# Autodesk Inventor assembly: ASY Beshkino_bio_tank
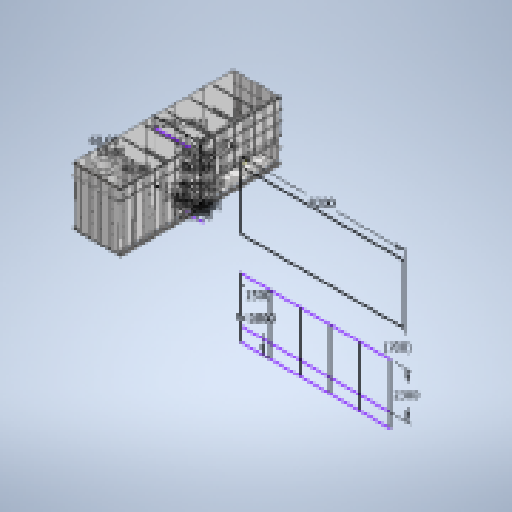
[picture p0: Inventor's stored thumbnail of the model, 512x512]
Saved by Autodesk Inventor 2025 (Build 290162010, 162A)
## iProperties
Created: 2024-07-21
Part Number: ASY Beshkino_bio_tank
Document SubType Name: Assembly
Designer: admin
Mass: 5.81287e+06 g
Surface Area: 2.77755e+06 cm^2
Volume: 3.12018e+06 cm^3
Density: 1.86299 g/cm^3
Author: admin
## Documents named in this file (46)
- C:\Users\DELL\YandexDisk-badmisterfox\домашниий пк\Inventor\BSH_Beshkino_bio_tank\ASY Beshkino_bio_tank.iam
- C:\Users\DELL\YandexDisk-badmisterfox\домашниий пк\Inventor\BSH_Beshkino_bio_tank\BSH 000 dim Beshkino_bio_tank.ipt
- C:\Users\DELL\YandexDisk-badmisterfox\домашниий пк\Inventor\BSH_Beshkino_bio_tank\BSH 011 floor.ipt
- C:\Users\DELL\YandexDisk-badmisterfox\домашниий пк\Inventor\BSH_Beshkino_bio_tank\BSH 021 rib floor.ipt
- C:\Users\DELL\YandexDisk-badmisterfox\домашниий пк\Inventor\BSH_Beshkino_bio_tank\BSH 022 rib board.ipt
- C:\Users\DELL\YandexDisk-badmisterfox\домашниий пк\Inventor\BSH_Beshkino_bio_tank\BSH 076 tube.ipt
- C:\Users\DELL\YandexDisk-badmisterfox\домашниий пк\Inventor\BSH_Beshkino_bio_tank\BSH 061 butt end.ipt
- C:\Users\DELL\YandexDisk-badmisterfox\домашниий пк\Inventor\BSH_Beshkino_bio_tank\BSH 041 board.ipt
- C:\Users\DELL\YandexDisk-badmisterfox\домашниий пк\Inventor\BSH_Beshkino_bio_tank\BSH 047 board.ipt
- C:\Users\DELL\YandexDisk-badmisterfox\домашниий пк\Inventor\BSH_Beshkino_bio_tank\BSH 045 back.ipt
- C:\Users\DELL\YandexDisk-badmisterfox\домашниий пк\Inventor\BSH_Beshkino_bio_tank\BSH 031 stringer floor.ipt
- C:\Users\DELL\YandexDisk-badmisterfox\домашниий пк\Inventor\BSH_Beshkino_bio_tank\BSH 036 stringer board 4.ipt
- C:\Users\DELL\YandexDisk-badmisterfox\домашниий пк\Inventor\BSH_Beshkino_bio_tank\BSH 032 stringer floor small.ipt
- C:\Users\DELL\YandexDisk-badmisterfox\домашниий пк\Inventor\BSH_Beshkino_bio_tank\BSH 039 stringer butt end in.ipt
- C:\Users\DELL\YandexDisk-badmisterfox\домашниий пк\Inventor\BSH_Beshkino_bio_tank\BSH 014 board cone.ipt
- C:\Users\DELL\YandexDisk-badmisterfox\домашниий пк\Inventor\BSH_Beshkino_bio_tank\BSH 051 sheet in.ipt
- C:\Users\DELL\YandexDisk-badmisterfox\домашниий пк\Inventor\BSH_Beshkino_bio_tank\BSH 071 amplifier in.ipt
- C:\Users\DELL\YandexDisk-badmisterfox\домашниий пк\Inventor\BSH_Beshkino_bio_tank\BSH 072 amplifier in.ipt
- C:\Users\DELL\YandexDisk-badmisterfox\домашниий пк\Inventor\BSH_Beshkino_bio_tank\BSH 012 floor.ipt
- C:\Users\DELL\YandexDisk-badmisterfox\домашниий пк\Inventor\BSH_Beshkino_bio_tank\BSH 016 cone.ipt
- C:\Users\DELL\YandexDisk-badmisterfox\домашниий пк\Inventor\BSH_Beshkino_bio_tank\BSH 013 floor.ipt
- C:\Users\DELL\YandexDisk-badmisterfox\домашниий пк\Inventor\BSH_Beshkino_bio_tank\BSH 015 board cone wall.ipt
- C:\Users\DELL\YandexDisk-badmisterfox\домашниий пк\Inventor\BSH_Beshkino_bio_tank\BSH 017 small detail floor.ipt
- C:\Users\DELL\YandexDisk-badmisterfox\домашниий пк\Inventor\BSH_Beshkino_bio_tank\BSH 038 stringer butt end.ipt
- C:\Users\DELL\YandexDisk-badmisterfox\домашниий пк\Inventor\BSH_Beshkino_bio_tank\BSH 053 sheet in.ipt
- C:\Users\DELL\YandexDisk-badmisterfox\домашниий пк\Inventor\BSH_Beshkino_bio_tank\BSH 044 board.ipt
- C:\Users\DELL\YandexDisk-badmisterfox\домашниий пк\Inventor\BSH_Beshkino_bio_tank\BSH 046 back.ipt
- C:\Users\DELL\YandexDisk-badmisterfox\домашниий пк\Inventor\BSH_Beshkino_bio_tank\BSH 042 board.ipt
- C:\Users\DELL\YandexDisk-badmisterfox\домашниий пк\Inventor\BSH_Beshkino_bio_tank\BSH 043 board.ipt
- C:\Users\DELL\YandexDisk-badmisterfox\домашниий пк\Inventor\BSH_Beshkino_bio_tank\BSH 052 sheet in.ipt
- C:\Users\DELL\YandexDisk-badmisterfox\домашниий пк\Inventor\BSH_Beshkino_bio_tank\BSH 023 rib butt end.ipt
- C:\Users\DELL\YandexDisk-badmisterfox\домашниий пк\Inventor\BSH_Beshkino_bio_tank\BSH 037 stringer board.ipt
- C:\Users\DELL\YandexDisk-badmisterfox\домашниий пк\Inventor\BSH_Beshkino_bio_tank\BSH 024 rib butt end in.ipt
- C:\Users\DELL\YandexDisk-badmisterfox\домашниий пк\Inventor\BSH_Beshkino_bio_tank\BSH 077 tube.ipt
- C:\Users\DELL\YandexDisk-badmisterfox\домашниий пк\Inventor\BSH_Beshkino_bio_tank\BSH 073 tube.ipt
- C:\Users\DELL\YandexDisk-badmisterfox\домашниий пк\Inventor\BSH_Beshkino_bio_tank\BSH 074 tube.ipt
- C:\Users\DELL\YandexDisk-badmisterfox\домашниий пк\Inventor\BSH_Beshkino_bio_tank\BSH 075 tube.ipt
- C:\Users\DELL\YandexDisk-badmisterfox\домашниий пк\Inventor\BSH_Beshkino_bio_tank\BSH 024 rib board short.ipt
- C:\Users\DELL\YandexDisk-badmisterfox\домашниий пк\Inventor\BSH_Beshkino_bio_tank\BSH 0363 stringer board 4.ipt
- C:\Users\DELL\YandexDisk-badmisterfox\домашниий пк\Inventor\BSH_Beshkino_bio_tank\BSH 022 rib floor 2.ipt
- C:\Users\DELL\YandexDisk-badmisterfox\домашниий пк\Inventor\BSH_Beshkino_bio_tank\BSH 033 stringer floor 3.ipt
- C:\Users\DELL\YandexDisk-badmisterfox\домашниий пк\Inventor\BSH_Beshkino_bio_tank\BSH 025 rib board cone.ipt
- C:\Users\DELL\YandexDisk-badmisterfox\домашниий пк\Inventor\BSH_Beshkino_bio_tank\ASY 080 barrel.iam
- C:\Users\DELL\YandexDisk-badmisterfox\домашниий пк\Inventor\BSH_Beshkino_bio_tank\BSH 0351 stringer board 3.ipt
- C:\Users\DELL\YandexDisk-badmisterfox\домашниий пк\Inventor\BSH_Beshkino_bio_tank\BSH 0341 stringer board 2.ipt
- C:\Users\DELL\YandexDisk-badmisterfox\домашниий пк\Inventor\BSH_Beshkino_bio_tank\BSH 014 board cone_CPY.ipt
## Components (129 placed, 48 different names)
1. BSH 000 dim Beshkino_bio_tank:1
2. BSH 076 tube:1 — Mate:1, Rigid:1, Mate:3, Mate:119, Flush:121, Flush:122, Mate:121, Flush:123
3. BSH 076 tube:2 — Mate:2, Rigid:1, Mate:4, Flush:3, Flush:4, Flush:124, Mate:132, Flush:128
4. BSH 011 floor:1 — Rigid:5, Rigid:83, Mate:77, Flush:18, Flush:19
5. BSH 011 floor:2 — Rigid:5, Rigid:82
6. BSH 011 floor:3 — Mate:5, Mate:6, Mate:7, Flush:4, Mate:10, Flush:5, Flush:11, Rigid:82, Mate:74, Mate:133
7. BSH 061 butt end:1 — Mate:10, Flush:5, Mate:11, Rigid:11, Mate:73, Mate:108, Mate:135, Flush:131, Mate:136
8. BSH 047 board:1 — Flush:11, Mate:73, Mate:74, Rigid:104, Mate:127, Flush:125, Flush:126, Mate:128, Flush:127
9. BSH 061 butt end:2 — Rigid:11, Rigid:53
10. BSH 021 rib floor:1 — Mate:4, Flush:3, Mate:5, Mate:6, Rigid:9, Rigid:109, Rigid:118, Rigid:122, Mate:120, Rigid:156
11. BSH 061 butt end:3 — Mate:113
12. BSH 061 butt end:4 — Rigid:53, Flush:112
13. BSH 014 board cone:1 — Mate:26, Rigid:57, Mate:30, Mate:80, Mate:83
14. BSH 061 butt end:5 — Mate:26, Mate:30, Mate:84, Flush:21, Mate:94, Mate:141
15. BSH 061 butt end:6 — Flush:8, Mate:40, Mate:111, Mate:137, Mate:138
16. BSH 014 board cone:2 — Rigid:57, Angle:1, Mate:49, Mate:50, Mate:64, Mate:71
17. BSH 036 stringer board 4:4 — Rigid:141
18. BSH 037 stringer board:1 — Rigid:141, Rigid:142
19. BSH 0363 stringer board 4:1 — Rigid:142, Rigid:143
20. BSH 051 sheet in:1 — Mate:84, Rigid:108, Mate:88, Mate:89, Mate:90, Mate:91, Mate:123
21. BSH 012 floor:1 — Rigid:66, Mate:42, Angle:1, Mate:49, Rigid:83, Mate:72, Mate:87
22. BSH 016 cone:1 — Mate:42, Mate:50, Mate:90
23. BSH 047 board:2 — Rigid:139
24. BSH 012 floor:2 — Rigid:66, Rigid:67, Mate:63, Mate:78, Mate:122
25. BSH 013 floor:1 — Rigid:67, Mate:40, Mate:81
26. BSH 045 back:1 — Rigid:90, Rigid:103
27. BSH 015 board cone wall:1 — Mate:71, Mate:72, Mate:85, Mate:86
28. BSH 017 small detail floor:1 — Mate:77, Flush:18, Flush:19
29. BSH 038 stringer butt end:1 — Mate:107, Mate:108, Rigid:128, Rigid:129, Rigid:130, Rigid:131
30. BSH 016 cone:2 — Mate:63, Mate:64, Mate:91
31. BSH 022 rib board:2 — Rigid:137, Mate:117, Flush:117
32. BSH 016 cone:3 — Mate:78, Mate:80, Mate:88
33. BSH 016 cone:4 — Mate:81, Mate:83, Mate:89
34. BSH 053 sheet in:1 — Rigid:107
35. BSH 044 board:1 — Rigid:90, Mate:85, Rigid:106
36. BSH 046 back:1 — Rigid:103, Flush:21, Mate:96, Flush:132, Mate:139
37. BSH 042 board:1 — Rigid:104, Rigid:105
38. BSH 043 board:1 — Rigid:105, Rigid:106
39. BSH 052 sheet in:1 — Rigid:107, Rigid:108, Mate:86, Mate:87
40. BSH 031 stringer floor:1 — Rigid:109, Rigid:147
41. BSH 032 stringer floor small:1 — Mate:131, Rigid:146
42. BSH 031 stringer floor:4 — Rigid:118
43. BSH 031 stringer floor:7 — Rigid:122
44. BSH 031 stringer floor:12 — Rigid:156
45. BSH 023 rib butt end:1 — Rigid:128, Mate:130
46. BSH 023 rib butt end:2 — Rigid:129
47. BSH 023 rib butt end:3 — Rigid:130
48. BSH 023 rib butt end:4 — Rigid:131
49. BSH 023 rib butt end:5
50. BSH 023 rib butt end:6
51. BSH 023 rib butt end:7
52. BSH 023 rib butt end:8 — Flush:129
53. BSH 022 rib board:3 — Rigid:138, Mate:128, Mate:129, Flush:127, Rigid:143
54. BSH 022 rib board:4 — Rigid:137
55. BSH 077 tube:1 — Mate:119, Flush:121, Flush:122, Mate:120, Mate:130
56. BSH 077 tube:2 — Mate:121, Flush:123, Flush:124, Mate:131, Flush:129
57. BSH 073 tube:1 — Mate:122, Mate:123, Mate:124
58. BSH 074 tube:1 — Mate:135, Flush:131, Mate:136
59. BSH 075 tube:2 — Mate:127, Flush:125, Flush:126, Mate:129, Mate:140
60. BSH 033 stringer floor 3:1 — Rigid:147
61. BSH 025 rib board cone:1 — Flush:130, Mate:134
62. ASY 080 barrel:1 [sub-assembly] — Mate:133
63. BSH 0351 stringer board 3:1 — Rigid:148
64. BSH 0341 stringer board 2:1 — Rigid:149
65. BSH 042 stringer floor:2 — Rigid:150
66. BSH 042 stringer floor:3 — Rigid:151
67. BSH 042 stringer floor:4 — Rigid:152
68. BSH 033 stringer floor 3:2 — Rigid:154
69. BSH 033 stringer floor 3:3 — Rigid:153
70. BSH 033 stringer floor 3:4 — Rigid:155
71. BSH 051 water tray:1 — Mate:139, Mate:140, Mate:141
72. BSH 041 board:1 — Mate:117, Flush:117, Rigid:139
73. BSH 041 board:2
74. BSH 041 board:3
75. BSH 041 board:4
76. BSH 041 board:5 — Mate:137, Flush:132, Mate:138
77. BSH 071 amplifier in:1 — Flush:22, Mate:94, Mate:96, Flush:24, Mate:97, Mate:124
78. BSH 072 amplifier in:1 — Flush:22, Mate:93, Flush:24
79. BSH 071 amplifier in:2
80. BSH 072 amplifier in:2
81. BSH 071 amplifier in:3
82. BSH 072 amplifier in:3
83. BSH 071 amplifier in:4
84. BSH 072 amplifier in:4
85. BSH 071 amplifier in:5
86. BSH 072 amplifier in:5
87. BSH 039 stringer butt end in:1 — Mate:23, Flush:112, Mate:113, Rigid:140
88. BSH 039 stringer butt end in:2
89. BSH 039 stringer butt end in:3
90. BSH 039 stringer butt end in:4
91. BSH 039 stringer butt end in:5
92. BSH 024 rib butt end in:1 — Rigid:140
93. BSH 024 rib butt end in:2
94. BSH 024 rib butt end in:3
95. BSH 024 rib butt end in:4
96. BSH 022 rib board:1 — Rigid:138
97. BSH 022 rib 2:36
98. BSH 022 rib 2:37
99. BSH 022 rib 2:38
100. BSH 022 rib 2:39
101. BSH 022 rib 2:40
102. BSH 022 rib 2:41
103. BSH 022 rib 2:42
104. BSH 022 rib 2:43 — Rigid:144
105. BSH 024 rib board short:1 — Rigid:144, Flush:130, Mate:134
106. BSH 024 rib board short:2
107. BSH 024 rib board short:3
108. BSH 024 rib board short:4
109. BSH 024 rib board short:5
110. BSH 024 rib board short:6 — Rigid:148, Rigid:149
111. BSH 021 rib floor:2 — Rigid:9
112. BSH 020 rib 1:4
113. BSH 020 rib 1:5
114. BSH 020 rib 1:6
115. BSH 020 rib 1:7 — Rigid:145
116. BSH 022 rib floor 2:1 — Rigid:146, Mate:132, Flush:128, Rigid:150, Rigid:151, Rigid:152
117. BSH 022 rib floor 2:2
118. BSH 022 rib floor 2:3
119. BSH 022 rib floor 2:4
120. BSH 022 rib floor 2:5
121. BSH 022 rib floor 2:6
122. BSH 020 rib 1:8 — Rigid:145
123. BSH 020 rib 1:9
124. BSH 020 rib 1:10
125. BSH 020 rib 1:11 — Rigid:153, Rigid:154, Rigid:155
126. BSH 038 stringer butt end:2 — Flush:111, Mate:111
127. BSH 038 stringer butt end:3
128. BSH 038 stringer butt end:4
129. BSH 038 stringer butt end:5
## Component patterns: (5 elements, first: BSH 041 board:1), (5 elements, first: BSH 071 amplifier in:1 + BSH 072 amplifier in:1), (5 elements, first: BSH 039 stringer butt end in:1), (4 elements, first: BSH 024 rib butt end in:1), (9 elements, first: BSH 022 rib board:1), (6 elements, first: BSH 024 rib board short:1), (5 elements, first: BSH 021 rib floor:2), (6 elements, first: BSH 022 rib floor 2:1), (4 elements, first: BSH 020 rib 1:8), (4 elements, first: BSH 038 stringer butt end:2)
## Relationships (141: Mate 65, WeldJoint 50, Flush 25, Angle 1)
- Mate:1: BSH 076 tube:1
- Mate:2: BSH 076 tube:2
- Rigid:1 [WeldJoint] (-2400 mm): BSH 076 tube:1 ↔ BSH 076 tube:2
- Mate:3: BSH 076 tube:1
- Mate:4: BSH 076 tube:2 ↔ BSH 021 rib floor:1
- Flush:3: BSH 076 tube:2 ↔ BSH 021 rib floor:1
- Mate:5: BSH 011 floor:3 ↔ BSH 021 rib floor:1
- Mate:6: BSH 011 floor:3 ↔ BSH 021 rib floor:1
- Rigid:5 [WeldJoint]: BSH 011 floor:1 ↔ BSH 011 floor:2
- Mate:7: BSH 011 floor:3
- Flush:4: BSH 076 tube:2 ↔ BSH 011 floor:3
- Rigid:9 [WeldJoint] (-500 mm): BSH 021 rib floor:1 ↔ BSH 021 rib floor:2
- Mate:10: BSH 011 floor:3 ↔ BSH 061 butt end:1
- Flush:5 (10 mm): BSH 011 floor:3 ↔ BSH 061 butt end:1
- Mate:11: BSH 061 butt end:1
- Rigid:11 [WeldJoint]: BSH 061 butt end:1 ↔ BSH 061 butt end:2
- Mate:23: BSH 039 stringer butt end in:1
- [WeldJoint]: BSH 061 butt end:3 ↔ BSH 061 butt end:4
- Rigid:53 [WeldJoint] (1500 mm): BSH 061 butt end:2 ↔ BSH 061 butt end:4
- [WeldJoint]: BSH 061 butt end:5 ↔ BSH 061 butt end:6
- Flush:8: BSH 061 butt end:6
- Mate:26: BSH 014 board cone:1 ↔ BSH 061 butt end:5
- Rigid:57 [WeldJoint]: BSH 014 board cone:1 ↔ BSH 014 board cone:2
- Mate:30: BSH 014 board cone:1 ↔ BSH 061 butt end:5
- Flush:11: BSH 011 floor:3 ↔ BSH 047 board:1
- Rigid:66 [WeldJoint]: BSH 012 floor:1 ↔ BSH 012 floor:2
- Rigid:67 [WeldJoint]: BSH 012 floor:2 ↔ BSH 013 floor:1
- Mate:40: BSH 061 butt end:6 ↔ BSH 013 floor:1
- Mate:42: BSH 012 floor:1 ↔ BSH 016 cone:1
- Angle:1 (132 deg): BSH 014 board cone:2 ↔ BSH 012 floor:1
- Mate:49: BSH 014 board cone:2 ↔ BSH 012 floor:1
- Mate:50: BSH 014 board cone:2 ↔ BSH 016 cone:1
- Mate:63: BSH 012 floor:2 ↔ BSH 016 cone:2
- Mate:64: BSH 014 board cone:2 ↔ BSH 016 cone:2
- Rigid:82 [WeldJoint]: BSH 011 floor:2 ↔ BSH 011 floor:3
- Rigid:83 [WeldJoint]: BSH 011 floor:1 ↔ BSH 012 floor:1
- Mate:71: BSH 014 board cone:2 ↔ BSH 015 board cone wall:1
- Mate:72: BSH 012 floor:1 ↔ BSH 015 board cone wall:1
- Mate:73: BSH 061 butt end:1 ↔ BSH 047 board:1
- Mate:74: BSH 011 floor:3 ↔ BSH 047 board:1
- Mate:77: BSH 011 floor:1 ↔ BSH 017 small detail floor:1
- Flush:18: BSH 011 floor:1 ↔ BSH 017 small detail floor:1
- Flush:19: BSH 011 floor:1 ↔ BSH 017 small detail floor:1
- Mate:78: BSH 012 floor:2 ↔ BSH 016 cone:3
- Mate:80: BSH 014 board cone:1 ↔ BSH 016 cone:3
- Mate:81: BSH 013 floor:1 ↔ BSH 016 cone:4
- Mate:83: BSH 014 board cone:1 ↔ BSH 016 cone:4
- Mate:84: BSH 061 butt end:5 ↔ BSH 051 sheet in:1
- Rigid:90 [WeldJoint]: BSH 045 back:1 ↔ BSH 044 board:1
- Mate:85: BSH 015 board cone wall:1 ↔ BSH 044 board:1
- Rigid:103 [WeldJoint]: BSH 045 back:1 ↔ BSH 046 back:1
- Rigid:104 [WeldJoint]: BSH 047 board:1 ↔ BSH 042 board:1
- Rigid:105 [WeldJoint]: BSH 042 board:1 ↔ BSH 043 board:1
- Rigid:106 [WeldJoint]: BSH 044 board:1 ↔ BSH 043 board:1
- Flush:21 (10 mm): BSH 061 butt end:5 ↔ BSH 046 back:1
- Rigid:107 [WeldJoint]: BSH 053 sheet in:1 ↔ BSH 052 sheet in:1
- Rigid:108 [WeldJoint]: BSH 051 sheet in:1 ↔ BSH 052 sheet in:1
- Mate:86: BSH 015 board cone wall:1 ↔ BSH 052 sheet in:1
- Mate:87: BSH 012 floor:1 ↔ BSH 052 sheet in:1
- Mate:88: BSH 051 sheet in:1 ↔ BSH 016 cone:3
- Mate:89: BSH 051 sheet in:1 ↔ BSH 016 cone:4
- Mate:90: BSH 051 sheet in:1 ↔ BSH 016 cone:1
- Mate:91: BSH 051 sheet in:1 ↔ BSH 016 cone:2
- Flush:22: BSH 071 amplifier in:1 ↔ BSH 072 amplifier in:1
- Mate:93: BSH 072 amplifier in:1
- Mate:94 (1000 mm): BSH 061 butt end:5 ↔ BSH 071 amplifier in:1
- Rigid:109 [WeldJoint] (2 mm): BSH 021 rib floor:1 ↔ BSH 031 stringer floor:1
- Rigid:118 [WeldJoint] (2 mm): BSH 021 rib floor:1 ↔ BSH 031 stringer floor:4
- Rigid:122 [WeldJoint] (2 mm): BSH 021 rib floor:1 ↔ BSH 031 stringer floor:7
- Mate:96 (100 mm): BSH 046 back:1 ↔ BSH 071 amplifier in:1
- Flush:24 (1000 mm): BSH 071 amplifier in:1 ↔ BSH 072 amplifier in:1
- Mate:97: BSH 071 amplifier in:1
- Mate:107: BSH 038 stringer butt end:1
- Mate:108: BSH 061 butt end:1 ↔ BSH 038 stringer butt end:1
- Rigid:128 [WeldJoint] (2 mm): BSH 038 stringer butt end:1 ↔ BSH 023 rib butt end:1
- Rigid:129 [WeldJoint] (2 mm): BSH 038 stringer butt end:1 ↔ BSH 023 rib butt end:2
- Rigid:130 [WeldJoint] (2 mm): BSH 038 stringer butt end:1 ↔ BSH 023 rib butt end:3
- Rigid:131 [WeldJoint] (2 mm): BSH 038 stringer butt end:1 ↔ BSH 023 rib butt end:4
- [WeldJoint] (2 mm): BSH 023 rib butt end:5 ↔ BSH 038 stringer butt end:2
- [WeldJoint] (2 mm): BSH 023 rib butt end:6 ↔ BSH 038 stringer butt end:2
- [WeldJoint] (2 mm): BSH 023 rib butt end:7 ↔ BSH 038 stringer butt end:2
- [WeldJoint] (2 mm): BSH 023 rib butt end:8 ↔ BSH 038 stringer butt end:2
- Flush:111: BSH 038 stringer butt end:2
- Mate:111: BSH 061 butt end:6 ↔ BSH 038 stringer butt end:2
- Flush:112 (171.5 mm): BSH 061 butt end:4 ↔ BSH 039 stringer butt end in:1
- Mate:113: BSH 061 butt end:3 ↔ BSH 039 stringer butt end in:1
- Rigid:137 [WeldJoint] (-436 mm): BSH 022 rib board:2 ↔ BSH 022 rib board:4
- Mate:117: BSH 022 rib board:2 ↔ BSH 041 board:1
- Flush:117 (-218 mm): BSH 022 rib board:2 ↔ BSH 041 board:1
- Rigid:138 [WeldJoint] (-500 mm): BSH 022 rib board:3 ↔ BSH 022 rib board:1
- Rigid:139 [WeldJoint]: BSH 047 board:2 ↔ BSH 041 board:1
- Rigid:140 [WeldJoint] (2 mm): BSH 039 stringer butt end in:1 ↔ BSH 024 rib butt end in:1
- Mate:119: BSH 076 tube:1 ↔ BSH 077 tube:1
- Flush:121: BSH 076 tube:1 ↔ BSH 077 tube:1
- Flush:122: BSH 076 tube:1 ↔ BSH 077 tube:1
- Mate:120 (117 mm): BSH 021 rib floor:1 ↔ BSH 077 tube:1
- Mate:121: BSH 076 tube:1 ↔ BSH 077 tube:2
- Flush:123: BSH 076 tube:1 ↔ BSH 077 tube:2
- Flush:124: BSH 076 tube:2 ↔ BSH 077 tube:2
- Mate:122: BSH 012 floor:2 ↔ BSH 073 tube:1
- Mate:123: BSH 051 sheet in:1 ↔ BSH 073 tube:1
- Mate:124: BSH 073 tube:1 ↔ BSH 071 amplifier in:1
- Rigid:141 [WeldJoint]: BSH 036 stringer board 4:4 ↔ BSH 037 stringer board:1
- Mate:127: BSH 047 board:1 ↔ BSH 075 tube:2
- Flush:125: BSH 047 board:1 ↔ BSH 075 tube:2
- Flush:126 (-40 mm): BSH 047 board:1 ↔ BSH 075 tube:2
- Mate:128: BSH 047 board:1 ↔ BSH 022 rib board:3
- Mate:129: BSH 022 rib board:3 ↔ BSH 075 tube:2
- Flush:127 (213.5 mm): BSH 047 board:1 ↔ BSH 022 rib board:3
- Rigid:142 [WeldJoint]: BSH 037 stringer board:1 ↔ BSH 0363 stringer board 4:1
- Rigid:143 [WeldJoint] (2 mm): BSH 0363 stringer board 4:1 ↔ BSH 022 rib board:3
- Rigid:144 [WeldJoint] (500 mm): BSH 022 rib 2:43 ↔ BSH 024 rib board short:1
- Mate:130: BSH 023 rib butt end:1 ↔ BSH 077 tube:1
- Mate:131: BSH 032 stringer floor small:1 ↔ BSH 077 tube:2
- Rigid:145 [WeldJoint] (500 mm): BSH 020 rib 1:7 ↔ BSH 020 rib 1:8
- Rigid:146 [WeldJoint] (2 mm): BSH 032 stringer floor small:1 ↔ BSH 022 rib floor 2:1
- Mate:132: BSH 076 tube:2 ↔ BSH 022 rib floor 2:1
- Flush:128: BSH 076 tube:2 ↔ BSH 022 rib floor 2:1
- Rigid:147 [WeldJoint] (-10 mm): BSH 031 stringer floor:1 ↔ BSH 033 stringer floor 3:1
- Flush:129: BSH 023 rib butt end:8 ↔ BSH 077 tube:2
- Mate:133: BSH 011 floor:3 ↔ ASY 080 barrel:1
- Flush:130: BSH 025 rib board cone:1 ↔ BSH 024 rib board short:1
- Mate:134: BSH 025 rib board cone:1 ↔ BSH 024 rib board short:1
- Rigid:148 [WeldJoint] (2 mm): BSH 0351 stringer board 3:1 ↔ BSH 024 rib board short:6
- Rigid:149 [WeldJoint] (2 mm): BSH 0341 stringer board 2:1 ↔ BSH 024 rib board short:6
- Mate:135: BSH 061 butt end:1 ↔ BSH 074 tube:1
- Flush:131: BSH 061 butt end:1 ↔ BSH 074 tube:1
- Mate:136: BSH 061 butt end:1 ↔ BSH 074 tube:1
- Rigid:150 [WeldJoint] (2 mm): BSH 042 stringer floor:2 ↔ BSH 022 rib floor 2:1
- Rigid:151 [WeldJoint] (2 mm): BSH 042 stringer floor:3 ↔ BSH 022 rib floor 2:1
- Rigid:152 [WeldJoint] (2 mm): BSH 042 stringer floor:4 ↔ BSH 022 rib floor 2:1
- Rigid:153 [WeldJoint]: BSH 033 stringer floor 3:3 ↔ BSH 020 rib 1:11
- Rigid:154 [WeldJoint] (2 mm): BSH 033 stringer floor 3:2 ↔ BSH 020 rib 1:11
- Rigid:155 [WeldJoint] (2 mm): BSH 033 stringer floor 3:4 ↔ BSH 020 rib 1:11
- Rigid:156 [WeldJoint] (2 mm): BSH 021 rib floor:1 ↔ BSH 031 stringer floor:12
- Mate:137: BSH 061 butt end:6 ↔ BSH 041 board:5
- Flush:132: BSH 046 back:1 ↔ BSH 041 board:5
- Mate:138: BSH 061 butt end:6 ↔ BSH 041 board:5
- Mate:139 (100 mm): BSH 046 back:1 ↔ BSH 051 water tray:1
- Mate:140: BSH 075 tube:2 ↔ BSH 051 water tray:1
- Mate:141: BSH 061 butt end:5 ↔ BSH 051 water tray:1
## Named parameters: d118_d31 = 0 mm, d124_d31 = 0 mm, d381_d380 = 2 mm, d382_d377 = 2 mm, d383_d378 = 2 mm, d384_d379 = 2 mm
